# Autodesk Inventor assembly: Intake 3
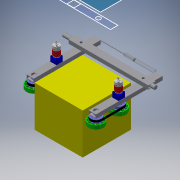
[picture p0: Inventor's stored thumbnail of the model, 180x180]
Saved by Autodesk Inventor 2018 (Build 220112000, 112)
## iProperties
Created: 2018-01-22
Part Number: Intake 3
Document SubType Name: Assembly
Designer: Apple
Author: Apple
## Documents named in this file (5)
- C:\Users\Apple\Documents\Inventor\2018 PowerUp\Cube Intake\Intake 3.iam
- C:\Users\Apple\Documents\Inventor\2018 PowerUp\Cube Intake\Intake 3 Arm.iam
- C:\Users\Apple\Documents\Inventor\2018 PowerUp\2018 power cube.ipt
- C:\Users\Apple\Documents\Inventor\2018 PowerUp\Cube Intake\Intake 3 Cross Bar.ipt
- C:\Users\Apple\Documents\Inventor\2018 PowerUp\Cube Intake\8in Cyl.iam
## Components (5 placed, 4 different names)
1. Intake 3 Cross Bar:1 — Mate:1, Mate:2, Mate:3, Angle:1, Angle:2
2. Intake 3 Arm:1 [sub-assembly] — Mate:1, Flush:1, Mate:5, Mate:6, Angle:2
3. Intake 3 Arm:2 [sub-assembly] — Mate:2, Flush:1, Mate:3, Mate:4, Mate:7, Angle:1, Power Cube to arms
4. 2018 power cube:1 — Power Cube to arms
5. 8in Cyl:1 [sub-assembly] — Mate:4, Mate:5, Mate:6, Mate:7
## Relationships (11: Mate 7, Flush 2, Angle 2)
- Mate:1: Intake 3 Cross Bar:1 ↔ Intake 3 Arm:1
- Mate:2: Intake 3 Cross Bar:1 ↔ Intake 3 Arm:2
- Flush:1: Intake 3 Arm:1 ↔ Intake 3 Arm:2
- Mate:3 (2.5 mm): Intake 3 Cross Bar:1 ↔ Intake 3 Arm:2
- Mate:4: Intake 3 Arm:2 ↔ 8in Cyl:1
- Mate:5: Intake 3 Arm:1 ↔ 8in Cyl:1
- Mate:6: Intake 3 Arm:1 ↔ 8in Cyl:1
- Mate:7: Intake 3 Arm:2 ↔ 8in Cyl:1
- Angle:1 (90 deg): Intake 3 Cross Bar:1 ↔ Intake 3 Arm:2
- Angle:2 (90 deg): Intake 3 Cross Bar:1 ↔ Intake 3 Arm:1
- Power Cube to arms [Flush] (-5 mm): Intake 3 Arm:2 ↔ 2018 power cube:1
